# Autodesk Inventor assembly: FRC Fixed Field 2018_sldasm
(part 3 of 4)
- C:\Users\CAD\Documents\GitHub\FIRST-ROBOTICS-2018-5436-CAD\Field\FIRST Power Up Field CAD\Body_1193_sldprt.ipt
- C:\Users\CAD\Documents\GitHub\FIRST-ROBOTICS-2018-5436-CAD\Field\FIRST Power Up Field CAD\Body_1194_sldprt.ipt
- C:\Users\CAD\Documents\GitHub\FIRST-ROBOTICS-2018-5436-CAD\Field\FIRST Power Up Field CAD\Body_1195_sldprt.ipt
- C:\Users\CAD\Documents\GitHub\FIRST-ROBOTICS-2018-5436-CAD\Field\FIRST Power Up Field CAD\Body_1196_sldprt.ipt
- C:\Users\CAD\Documents\GitHub\FIRST-ROBOTICS-2018-5436-CAD\Field\FIRST Power Up Field CAD\Body_1197_sldprt.ipt
- C:\Users\CAD\Documents\GitHub\FIRST-ROBOTICS-2018-5436-CAD\Field\FIRST Power Up Field CAD\Body_1198_sldprt.ipt
- C:\Users\CAD\Documents\GitHub\FIRST-ROBOTICS-2018-5436-CAD\Field\FIRST Power Up Field CAD\Body_1199_sldprt.ipt
- C:\Users\CAD\Documents\GitHub\FIRST-ROBOTICS-2018-5436-CAD\Field\FIRST Power Up Field CAD\Body_1200_sldprt.ipt
- C:\Users\CAD\Documents\GitHub\FIRST-ROBOTICS-2018-5436-CAD\Field\FIRST Power Up Field CAD\Body_1201_sldprt.ipt
- C:\Users\CAD\Documents\GitHub\FIRST-ROBOTICS-2018-5436-CAD\Field\FIRST Power Up Field CAD\Body_1202_sldprt.ipt
- C:\Users\CAD\Documents\GitHub\FIRST-ROBOTICS-2018-5436-CAD\Field\FIRST Power Up Field CAD\Body_1203_sldprt.ipt
- C:\Users\CAD\Documents\GitHub\FIRST-ROBOTICS-2018-5436-CAD\Field\FIRST Power Up Field CAD\Body_1204_sldprt.ipt
- C:\Users\CAD\Documents\GitHub\FIRST-ROBOTICS-2018-5436-CAD\Field\FIRST Power Up Field CAD\Body_1205_sldprt.ipt
- C:\Users\CAD\Documents\GitHub\FIRST-ROBOTICS-2018-5436-CAD\Field\FIRST Power Up Field CAD\Body_1206_sldprt.ipt
- C:\Users\CAD\Documents\GitHub\FIRST-ROBOTICS-2018-5436-CAD\Field\FIRST Power Up Field CAD\Body_1207_sldprt.ipt
- C:\Users\CAD\Documents\GitHub\FIRST-ROBOTICS-2018-5436-CAD\Field\FIRST Power Up Field CAD\Body_1208_sldprt.ipt
- C:\Users\CAD\Documents\GitHub\FIRST-ROBOTICS-2018-5436-CAD\Field\FIRST Power Up Field CAD\Body_1209_sldprt.ipt
- C:\Users\CAD\Documents\GitHub\FIRST-ROBOTICS-2018-5436-CAD\Field\FIRST Power Up Field CAD\Body_1210_sldprt.ipt
- C:\Users\CAD\Documents\GitHub\FIRST-ROBOTICS-2018-5436-CAD\Field\FIRST Power Up Field CAD\Body_1211_sldprt.ipt
- C:\Users\CAD\Documents\GitHub\FIRST-ROBOTICS-2018-5436-CAD\Field\FIRST Power Up Field CAD\Body_1212_sldprt.ipt
- C:\Users\CAD\Documents\GitHub\FIRST-ROBOTICS-2018-5436-CAD\Field\FIRST Power Up Field CAD\Body_1213_sldprt.ipt
- C:\Users\CAD\Documents\GitHub\FIRST-ROBOTICS-2018-5436-CAD\Field\FIRST Power Up Field CAD\Body_1214_sldprt.ipt
- C:\Users\CAD\Documents\GitHub\FIRST-ROBOTICS-2018-5436-CAD\Field\FIRST Power Up Field CAD\Body_1215_sldprt.ipt
- C:\Users\CAD\Documents\GitHub\FIRST-ROBOTICS-2018-5436-CAD\Field\FIRST Power Up Field CAD\Body_1216_sldprt.ipt
- C:\Users\CAD\Documents\GitHub\FIRST-ROBOTICS-2018-5436-CAD\Field\FIRST Power Up Field CAD\Body_1217_sldprt.ipt
- C:\Users\CAD\Documents\GitHub\FIRST-ROBOTICS-2018-5436-CAD\Field\FIRST Power Up Field CAD\Body_1218_sldprt.ipt
- C:\Users\CAD\Documents\GitHub\FIRST-ROBOTICS-2018-5436-CAD\Field\FIRST Power Up Field CAD\Body_1219_sldprt.ipt
- C:\Users\CAD\Documents\GitHub\FIRST-ROBOTICS-2018-5436-CAD\Field\FIRST Power Up Field CAD\Body_1220_sldprt.ipt
- C:\Users\CAD\Documents\GitHub\FIRST-ROBOTICS-2018-5436-CAD\Field\FIRST Power Up Field CAD\Body_1221_sldprt.ipt
- C:\Users\CAD\Documents\GitHub\FIRST-ROBOTICS-2018-5436-CAD\Field\FIRST Power Up Field CAD\Body_1222_sldprt.ipt
- C:\Users\CAD\Documents\GitHub\FIRST-ROBOTICS-2018-5436-CAD\Field\FIRST Power Up Field CAD\Body_1223_sldprt.ipt
- C:\Users\CAD\Documents\GitHub\FIRST-ROBOTICS-2018-5436-CAD\Field\FIRST Power Up Field CAD\Body_1224_sldprt.ipt
- C:\Users\CAD\Documents\GitHub\FIRST-ROBOTICS-2018-5436-CAD\Field\FIRST Power Up Field CAD\Body_1225_sldprt.ipt
- C:\Users\CAD\Documents\GitHub\FIRST-ROBOTICS-2018-5436-CAD\Field\FIRST Power Up Field CAD\Body_1226_sldprt.ipt
- C:\Users\CAD\Documents\GitHub\FIRST-ROBOTICS-2018-5436-CAD\Field\FIRST Power Up Field CAD\Body_1227_sldprt.ipt
- C:\Users\CAD\Documents\GitHub\FIRST-ROBOTICS-2018-5436-CAD\Field\FIRST Power Up Field CAD\Body_1228_sldprt.ipt
- C:\Users\CAD\Documents\GitHub\FIRST-ROBOTICS-2018-5436-CAD\Field\FIRST Power Up Field CAD\Body_1229_sldprt.ipt
- C:\Users\CAD\Documents\GitHub\FIRST-ROBOTICS-2018-5436-CAD\Field\FIRST Power Up Field CAD\Body_1230_sldprt.ipt
- C:\Users\CAD\Documents\GitHub\FIRST-ROBOTICS-2018-5436-CAD\Field\FIRST Power Up Field CAD\Body_1231_sldprt.ipt
- C:\Users\CAD\Documents\GitHub\FIRST-ROBOTICS-2018-5436-CAD\Field\FIRST Power Up Field CAD\Body_1232_sldprt.ipt
- C:\Users\CAD\Documents\GitHub\FIRST-ROBOTICS-2018-5436-CAD\Field\FIRST Power Up Field CAD\Body_1233_sldprt.ipt
- C:\Users\CAD\Documents\GitHub\FIRST-ROBOTICS-2018-5436-CAD\Field\FIRST Power Up Field CAD\Body_1234_sldprt.ipt
- C:\Users\CAD\Documents\GitHub\FIRST-ROBOTICS-2018-5436-CAD\Field\FIRST Power Up Field CAD\Body_1235_sldprt.ipt
- C:\Users\CAD\Documents\GitHub\FIRST-ROBOTICS-2018-5436-CAD\Field\FIRST Power Up Field CAD\Body_1236_sldprt.ipt
- C:\Users\CAD\Documents\GitHub\FIRST-ROBOTICS-2018-5436-CAD\Field\FIRST Power Up Field CAD\Body_1237_sldprt.ipt
- C:\Users\CAD\Documents\GitHub\FIRST-ROBOTICS-2018-5436-CAD\Field\FIRST Power Up Field CAD\Body_1238_sldprt.ipt
- C:\Users\CAD\Documents\GitHub\FIRST-ROBOTICS-2018-5436-CAD\Field\FIRST Power Up Field CAD\Body_1239_sldprt.ipt
- C:\Users\CAD\Documents\GitHub\FIRST-ROBOTICS-2018-5436-CAD\Field\FIRST Power Up Field CAD\Body_1240_sldprt.ipt
- C:\Users\CAD\Documents\GitHub\FIRST-ROBOTICS-2018-5436-CAD\Field\FIRST Power Up Field CAD\Body_1241_sldprt.ipt
- C:\Users\CAD\Documents\GitHub\FIRST-ROBOTICS-2018-5436-CAD\Field\FIRST Power Up Field CAD\Body_1242_sldprt.ipt
- C:\Users\CAD\Documents\GitHub\FIRST-ROBOTICS-2018-5436-CAD\Field\FIRST Power Up Field CAD\Body_1243_sldprt.ipt
- C:\Users\CAD\Documents\GitHub\FIRST-ROBOTICS-2018-5436-CAD\Field\FIRST Power Up Field CAD\Body_1244_sldprt.ipt
- C:\Users\CAD\Documents\GitHub\FIRST-ROBOTICS-2018-5436-CAD\Field\FIRST Power Up Field CAD\Body_1245_sldprt.ipt
- C:\Users\CAD\Documents\GitHub\FIRST-ROBOTICS-2018-5436-CAD\Field\FIRST Power Up Field CAD\Body_1246_sldprt.ipt
- C:\Users\CAD\Documents\GitHub\FIRST-ROBOTICS-2018-5436-CAD\Field\FIRST Power Up Field CAD\Body_1247_sldprt.ipt
- C:\Users\CAD\Documents\GitHub\FIRST-ROBOTICS-2018-5436-CAD\Field\FIRST Power Up Field CAD\Body_1248_sldprt.ipt
- C:\Users\CAD\Documents\GitHub\FIRST-ROBOTICS-2018-5436-CAD\Field\FIRST Power Up Field CAD\Body_1249_sldprt.ipt
- C:\Users\CAD\Documents\GitHub\FIRST-ROBOTICS-2018-5436-CAD\Field\FIRST Power Up Field CAD\Body_1250_sldprt.ipt
- C:\Users\CAD\Documents\GitHub\FIRST-ROBOTICS-2018-5436-CAD\Field\FIRST Power Up Field CAD\Body_1251_sldprt.ipt
- C:\Users\CAD\Documents\GitHub\FIRST-ROBOTICS-2018-5436-CAD\Field\FIRST Power Up Field CAD\Body_1252_sldprt.ipt
- C:\Users\CAD\Documents\GitHub\FIRST-ROBOTICS-2018-5436-CAD\Field\FIRST Power Up Field CAD\Body_1253_sldprt.ipt
- C:\Users\CAD\Documents\GitHub\FIRST-ROBOTICS-2018-5436-CAD\Field\FIRST Power Up Field CAD\Body_1254_sldprt.ipt
- C:\Users\CAD\Documents\GitHub\FIRST-ROBOTICS-2018-5436-CAD\Field\FIRST Power Up Field CAD\Body_1255_sldprt.ipt
- C:\Users\CAD\Documents\GitHub\FIRST-ROBOTICS-2018-5436-CAD\Field\FIRST Power Up Field CAD\Body_1256_sldprt.ipt
- C:\Users\CAD\Documents\GitHub\FIRST-ROBOTICS-2018-5436-CAD\Field\FIRST Power Up Field CAD\Body_1257_sldprt.ipt
- C:\Users\CAD\Documents\GitHub\FIRST-ROBOTICS-2018-5436-CAD\Field\FIRST Power Up Field CAD\Body_1258_sldprt.ipt
- C:\Users\CAD\Documents\GitHub\FIRST-ROBOTICS-2018-5436-CAD\Field\FIRST Power Up Field CAD\Body_1259_sldprt.ipt
- C:\Users\CAD\Documents\GitHub\FIRST-ROBOTICS-2018-5436-CAD\Field\FIRST Power Up Field CAD\Body_1260_sldprt.ipt
- C:\Users\CAD\Documents\GitHub\FIRST-ROBOTICS-2018-5436-CAD\Field\FIRST Power Up Field CAD\Body_1261_sldprt.ipt
- C:\Users\CAD\Documents\GitHub\FIRST-ROBOTICS-2018-5436-CAD\Field\FIRST Power Up Field CAD\Body_1262_sldprt.ipt
- C:\Users\CAD\Documents\GitHub\FIRST-ROBOTICS-2018-5436-CAD\Field\FIRST Power Up Field CAD\Body_1263_sldprt.ipt
- C:\Users\CAD\Documents\GitHub\FIRST-ROBOTICS-2018-5436-CAD\Field\FIRST Power Up Field CAD\Body_1264_sldprt.ipt
- C:\Users\CAD\Documents\GitHub\FIRST-ROBOTICS-2018-5436-CAD\Field\FIRST Power Up Field CAD\Body_1265_sldprt.ipt
- C:\Users\CAD\Documents\GitHub\FIRST-ROBOTICS-2018-5436-CAD\Field\FIRST Power Up Field CAD\Body_1266_sldprt.ipt
- C:\Users\CAD\Documents\GitHub\FIRST-ROBOTICS-2018-5436-CAD\Field\FIRST Power Up Field CAD\Body_1267_sldprt.ipt
- C:\Users\CAD\Documents\GitHub\FIRST-ROBOTICS-2018-5436-CAD\Field\FIRST Power Up Field CAD\Body_1268_sldprt.ipt
- C:\Users\CAD\Documents\GitHub\FIRST-ROBOTICS-2018-5436-CAD\Field\FIRST Power Up Field CAD\Body_1269_sldprt.ipt
- C:\Users\CAD\Documents\GitHub\FIRST-ROBOTICS-2018-5436-CAD\Field\FIRST Power Up Field CAD\Body_1270_sldprt.ipt
- C:\Users\CAD\Documents\GitHub\FIRST-ROBOTICS-2018-5436-CAD\Field\FIRST Power Up Field CAD\Body_1271_sldprt.ipt
- C:\Users\CAD\Documents\GitHub\FIRST-ROBOTICS-2018-5436-CAD\Field\FIRST Power Up Field CAD\Body_1272_sldprt.ipt
- C:\Users\CAD\Documents\GitHub\FIRST-ROBOTICS-2018-5436-CAD\Field\FIRST Power Up Field CAD\Body_1273_sldprt.ipt
- C:\Users\CAD\Documents\GitHub\FIRST-ROBOTICS-2018-5436-CAD\Field\FIRST Power Up Field CAD\Body_1274_sldprt.ipt
- C:\Users\CAD\Documents\GitHub\FIRST-ROBOTICS-2018-5436-CAD\Field\FIRST Power Up Field CAD\Body_1275_sldprt.ipt
- C:\Users\CAD\Documents\GitHub\FIRST-ROBOTICS-2018-5436-CAD\Field\FIRST Power Up Field CAD\Body_1276_sldprt.ipt
- C:\Users\CAD\Documents\GitHub\FIRST-ROBOTICS-2018-5436-CAD\Field\FIRST Power Up Field CAD\Body_1277_sldprt.ipt
- C:\Users\CAD\Documents\GitHub\FIRST-ROBOTICS-2018-5436-CAD\Field\FIRST Power Up Field CAD\Body_1278_sldprt.ipt
- C:\Users\CAD\Documents\GitHub\FIRST-ROBOTICS-2018-5436-CAD\Field\FIRST Power Up Field CAD\Body_1279_sldprt.ipt
- C:\Users\CAD\Documents\GitHub\FIRST-ROBOTICS-2018-5436-CAD\Field\FIRST Power Up Field CAD\Body_1280_sldprt.ipt
- C:\Users\CAD\Documents\GitHub\FIRST-ROBOTICS-2018-5436-CAD\Field\FIRST Power Up Field CAD\Body_1281_sldprt.ipt
- C:\Users\CAD\Documents\GitHub\FIRST-ROBOTICS-2018-5436-CAD\Field\FIRST Power Up Field CAD\Body_1282_sldprt.ipt
- C:\Users\CAD\Documents\GitHub\FIRST-ROBOTICS-2018-5436-CAD\Field\FIRST Power Up Field CAD\Body_1283_sldprt.ipt
- C:\Users\CAD\Documents\GitHub\FIRST-ROBOTICS-2018-5436-CAD\Field\FIRST Power Up Field CAD\Body_1284_sldprt.ipt
- C:\Users\CAD\Documents\GitHub\FIRST-ROBOTICS-2018-5436-CAD\Field\FIRST Power Up Field CAD\Body_1285_sldprt.ipt
- C:\Users\CAD\Documents\GitHub\FIRST-ROBOTICS-2018-5436-CAD\Field\FIRST Power Up Field CAD\Body_1286_sldprt.ipt
- C:\Users\CAD\Documents\GitHub\FIRST-ROBOTICS-2018-5436-CAD\Field\FIRST Power Up Field CAD\Body_1287_sldprt.ipt
- C:\Users\CAD\Documents\GitHub\FIRST-ROBOTICS-2018-5436-CAD\Field\FIRST Power Up Field CAD\Body_1288_sldprt.ipt
- C:\Users\CAD\Documents\GitHub\FIRST-ROBOTICS-2018-5436-CAD\Field\FIRST Power Up Field CAD\Body_1289_sldprt.ipt
- C:\Users\CAD\Documents\GitHub\FIRST-ROBOTICS-2018-5436-CAD\Field\FIRST Power Up Field CAD\Body_1290_sldprt.ipt
- C:\Users\CAD\Documents\GitHub\FIRST-ROBOTICS-2018-5436-CAD\Field\FIRST Power Up Field CAD\Body_1291_sldprt.ipt
- C:\Users\CAD\Documents\GitHub\FIRST-ROBOTICS-2018-5436-CAD\Field\FIRST Power Up Field CAD\Body_1292_sldprt.ipt
- C:\Users\CAD\Documents\GitHub\FIRST-ROBOTICS-2018-5436-CAD\Field\FIRST Power Up Field CAD\Body_1293_sldprt.ipt
- C:\Users\CAD\Documents\GitHub\FIRST-ROBOTICS-2018-5436-CAD\Field\FIRST Power Up Field CAD\Body_1294_sldprt.ipt
- C:\Users\CAD\Documents\GitHub\FIRST-ROBOTICS-2018-5436-CAD\Field\FIRST Power Up Field CAD\Body_1295_sldprt.ipt
- C:\Users\CAD\Documents\GitHub\FIRST-ROBOTICS-2018-5436-CAD\Field\FIRST Power Up Field CAD\Body_1296_sldprt.ipt
- C:\Users\CAD\Documents\GitHub\FIRST-ROBOTICS-2018-5436-CAD\Field\FIRST Power Up Field CAD\Body_1297_sldprt.ipt
- C:\Users\CAD\Documents\GitHub\FIRST-ROBOTICS-2018-5436-CAD\Field\FIRST Power Up Field CAD\Body_1298_sldprt.ipt
- C:\Users\CAD\Documents\GitHub\FIRST-ROBOTICS-2018-5436-CAD\Field\FIRST Power Up Field CAD\Body_1299_sldprt.ipt
- C:\Users\CAD\Documents\GitHub\FIRST-ROBOTICS-2018-5436-CAD\Field\FIRST Power Up Field CAD\Body_1300_sldprt.ipt
- C:\Users\CAD\Documents\GitHub\FIRST-ROBOTICS-2018-5436-CAD\Field\FIRST Power Up Field CAD\Body_1301_sldprt.ipt
- C:\Users\CAD\Documents\GitHub\FIRST-ROBOTICS-2018-5436-CAD\Field\FIRST Power Up Field CAD\Body_1302_sldprt.ipt
- C:\Users\CAD\Documents\GitHub\FIRST-ROBOTICS-2018-5436-CAD\Field\FIRST Power Up Field CAD\Body_1303_sldprt.ipt
- C:\Users\CAD\Documents\GitHub\FIRST-ROBOTICS-2018-5436-CAD\Field\FIRST Power Up Field CAD\Body_1304_sldprt.ipt
- C:\Users\CAD\Documents\GitHub\FIRST-ROBOTICS-2018-5436-CAD\Field\FIRST Power Up Field CAD\Body_1305_sldprt.ipt
- C:\Users\CAD\Documents\GitHub\FIRST-ROBOTICS-2018-5436-CAD\Field\FIRST Power Up Field CAD\Body_1306_sldprt.ipt
- C:\Users\CAD\Documents\GitHub\FIRST-ROBOTICS-2018-5436-CAD\Field\FIRST Power Up Field CAD\Body_1307_sldprt.ipt
- C:\Users\CAD\Documents\GitHub\FIRST-ROBOTICS-2018-5436-CAD\Field\FIRST Power Up Field CAD\Body_1308_sldprt.ipt
- C:\Users\CAD\Documents\GitHub\FIRST-ROBOTICS-2018-5436-CAD\Field\FIRST Power Up Field CAD\Body_1309_sldprt.ipt
- C:\Users\CAD\Documents\GitHub\FIRST-ROBOTICS-2018-5436-CAD\Field\FIRST Power Up Field CAD\Body_1310_sldprt.ipt
- C:\Users\CAD\Documents\GitHub\FIRST-ROBOTICS-2018-5436-CAD\Field\FIRST Power Up Field CAD\Body_1311_sldprt.ipt
- C:\Users\CAD\Documents\GitHub\FIRST-ROBOTICS-2018-5436-CAD\Field\FIRST Power Up Field CAD\Body_1312_sldprt.ipt
- C:\Users\CAD\Documents\GitHub\FIRST-ROBOTICS-2018-5436-CAD\Field\FIRST Power Up Field CAD\Body_1313_sldprt.ipt
- C:\Users\CAD\Documents\GitHub\FIRST-ROBOTICS-2018-5436-CAD\Field\FIRST Power Up Field CAD\Body_1314_sldprt.ipt
- C:\Users\CAD\Documents\GitHub\FIRST-ROBOTICS-2018-5436-CAD\Field\FIRST Power Up Field CAD\Body_1315_sldprt.ipt
- C:\Users\CAD\Documents\GitHub\FIRST-ROBOTICS-2018-5436-CAD\Field\FIRST Power Up Field CAD\Body_1316_sldprt.ipt
- C:\Users\CAD\Documents\GitHub\FIRST-ROBOTICS-2018-5436-CAD\Field\FIRST Power Up Field CAD\Body_1317_sldprt.ipt
- C:\Users\CAD\Documents\GitHub\FIRST-ROBOTICS-2018-5436-CAD\Field\FIRST Power Up Field CAD\Body_1318_sldprt.ipt
- C:\Users\CAD\Documents\GitHub\FIRST-ROBOTICS-2018-5436-CAD\Field\FIRST Power Up Field CAD\Body_1319_sldprt.ipt
- C:\Users\CAD\Documents\GitHub\FIRST-ROBOTICS-2018-5436-CAD\Field\FIRST Power Up Field CAD\Body_1320_sldprt.ipt
- C:\Users\CAD\Documents\GitHub\FIRST-ROBOTICS-2018-5436-CAD\Field\FIRST Power Up Field CAD\Body_1321_sldprt.ipt
- C:\Users\CAD\Documents\GitHub\FIRST-ROBOTICS-2018-5436-CAD\Field\FIRST Power Up Field CAD\Body_1322_sldprt.ipt
- C:\Users\CAD\Documents\GitHub\FIRST-ROBOTICS-2018-5436-CAD\Field\FIRST Power Up Field CAD\Body_1323_sldprt.ipt
- C:\Users\CAD\Documents\GitHub\FIRST-ROBOTICS-2018-5436-CAD\Field\FIRST Power Up Field CAD\Body_1324_sldprt.ipt
- C:\Users\CAD\Documents\GitHub\FIRST-ROBOTICS-2018-5436-CAD\Field\FIRST Power Up Field CAD\Body_1325_sldprt.ipt
- C:\Users\CAD\Documents\GitHub\FIRST-ROBOTICS-2018-5436-CAD\Field\FIRST Power Up Field CAD\Body_1326_sldprt.ipt
- C:\Users\CAD\Documents\GitHub\FIRST-ROBOTICS-2018-5436-CAD\Field\FIRST Power Up Field CAD\Body_1327_sldprt.ipt
- C:\Users\CAD\Documents\GitHub\FIRST-ROBOTICS-2018-5436-CAD\Field\FIRST Power Up Field CAD\Body_1328_sldprt.ipt
- C:\Users\CAD\Documents\GitHub\FIRST-ROBOTICS-2018-5436-CAD\Field\FIRST Power Up Field CAD\Body_1329_sldprt.ipt
- C:\Users\CAD\Documents\GitHub\FIRST-ROBOTICS-2018-5436-CAD\Field\FIRST Power Up Field CAD\Body_1330_sldprt.ipt
- C:\Users\CAD\Documents\GitHub\FIRST-ROBOTICS-2018-5436-CAD\Field\FIRST Power Up Field CAD\Body_1331_sldprt.ipt
- C:\Users\CAD\Documents\GitHub\FIRST-ROBOTICS-2018-5436-CAD\Field\FIRST Power Up Field CAD\Body_1332_sldprt.ipt
- C:\Users\CAD\Documents\GitHub\FIRST-ROBOTICS-2018-5436-CAD\Field\FIRST Power Up Field CAD\Body_1333_sldprt.ipt
- C:\Users\CAD\Documents\GitHub\FIRST-ROBOTICS-2018-5436-CAD\Field\FIRST Power Up Field CAD\Body_1334_sldprt.ipt
- C:\Users\CAD\Documents\GitHub\FIRST-ROBOTICS-2018-5436-CAD\Field\FIRST Power Up Field CAD\Body_1335_sldprt.ipt
- C:\Users\CAD\Documents\GitHub\FIRST-ROBOTICS-2018-5436-CAD\Field\FIRST Power Up Field CAD\Body_1336_sldprt.ipt
- C:\Users\CAD\Documents\GitHub\FIRST-ROBOTICS-2018-5436-CAD\Field\FIRST Power Up Field CAD\Body_1337_sldprt.ipt
- C:\Users\CAD\Documents\GitHub\FIRST-ROBOTICS-2018-5436-CAD\Field\FIRST Power Up Field CAD\Body_1338_sldprt.ipt
- C:\Users\CAD\Documents\GitHub\FIRST-ROBOTICS-2018-5436-CAD\Field\FIRST Power Up Field CAD\Body_1339_sldprt.ipt
- C:\Users\CAD\Documents\GitHub\FIRST-ROBOTICS-2018-5436-CAD\Field\FIRST Power Up Field CAD\Body_1340_sldprt.ipt
- C:\Users\CAD\Documents\GitHub\FIRST-ROBOTICS-2018-5436-CAD\Field\FIRST Power Up Field CAD\Body_1341_sldprt.ipt
- C:\Users\CAD\Documents\GitHub\FIRST-ROBOTICS-2018-5436-CAD\Field\FIRST Power Up Field CAD\Body_1342_sldprt.ipt
- C:\Users\CAD\Documents\GitHub\FIRST-ROBOTICS-2018-5436-CAD\Field\FIRST Power Up Field CAD\Body_1343_sldprt.ipt
- C:\Users\CAD\Documents\GitHub\FIRST-ROBOTICS-2018-5436-CAD\Field\FIRST Power Up Field CAD\Body_1344_sldprt.ipt
- C:\Users\CAD\Documents\GitHub\FIRST-ROBOTICS-2018-5436-CAD\Field\FIRST Power Up Field CAD\Body_1345_sldprt.ipt
- C:\Users\CAD\Documents\GitHub\FIRST-ROBOTICS-2018-5436-CAD\Field\FIRST Power Up Field CAD\Body_1346_sldprt.ipt
- C:\Users\CAD\Documents\GitHub\FIRST-ROBOTICS-2018-5436-CAD\Field\FIRST Power Up Field CAD\Body_1347_sldprt.ipt
- C:\Users\CAD\Documents\GitHub\FIRST-ROBOTICS-2018-5436-CAD\Field\FIRST Power Up Field CAD\Body_1348_sldprt.ipt
- C:\Users\CAD\Documents\GitHub\FIRST-ROBOTICS-2018-5436-CAD\Field\FIRST Power Up Field CAD\Body_1349_sldprt.ipt
- C:\Users\CAD\Documents\GitHub\FIRST-ROBOTICS-2018-5436-CAD\Field\FIRST Power Up Field CAD\Body_1350_sldprt.ipt
- C:\Users\CAD\Documents\GitHub\FIRST-ROBOTICS-2018-5436-CAD\Field\FIRST Power Up Field CAD\Body_1351_sldprt.ipt
- C:\Users\CAD\Documents\GitHub\FIRST-ROBOTICS-2018-5436-CAD\Field\FIRST Power Up Field CAD\Body_1352_sldprt.ipt
- C:\Users\CAD\Documents\GitHub\FIRST-ROBOTICS-2018-5436-CAD\Field\FIRST Power Up Field CAD\Body_1353_sldprt.ipt
- C:\Users\CAD\Documents\GitHub\FIRST-ROBOTICS-2018-5436-CAD\Field\FIRST Power Up Field CAD\Body_1354_sldprt.ipt
- C:\Users\CAD\Documents\GitHub\FIRST-ROBOTICS-2018-5436-CAD\Field\FIRST Power Up Field CAD\Body_1355_sldprt.ipt
- C:\Users\CAD\Documents\GitHub\FIRST-ROBOTICS-2018-5436-CAD\Field\FIRST Power Up Field CAD\Body_1356_sldprt.ipt
- C:\Users\CAD\Documents\GitHub\FIRST-ROBOTICS-2018-5436-CAD\Field\FIRST Power Up Field CAD\Body_1357_sldprt.ipt
- C:\Users\CAD\Documents\GitHub\FIRST-ROBOTICS-2018-5436-CAD\Field\FIRST Power Up Field CAD\Body_1358_sldprt.ipt
- C:\Users\CAD\Documents\GitHub\FIRST-ROBOTICS-2018-5436-CAD\Field\FIRST Power Up Field CAD\Body_1359_sldprt.ipt
- C:\Users\CAD\Documents\GitHub\FIRST-ROBOTICS-2018-5436-CAD\Field\FIRST Power Up Field CAD\Body_1360_sldprt.ipt
- C:\Users\CAD\Documents\GitHub\FIRST-ROBOTICS-2018-5436-CAD\Field\FIRST Power Up Field CAD\Body_1361_sldprt.ipt
- C:\Users\CAD\Documents\GitHub\FIRST-ROBOTICS-2018-5436-CAD\Field\FIRST Power Up Field CAD\Body_1362_sldprt.ipt
- C:\Users\CAD\Documents\GitHub\FIRST-ROBOTICS-2018-5436-CAD\Field\FIRST Power Up Field CAD\Body_1363_sldprt.ipt
- C:\Users\CAD\Documents\GitHub\FIRST-ROBOTICS-2018-5436-CAD\Field\FIRST Power Up Field CAD\Body_1364_sldprt.ipt
- C:\Users\CAD\Documents\GitHub\FIRST-ROBOTICS-2018-5436-CAD\Field\FIRST Power Up Field CAD\Body_1365_sldprt.ipt
- C:\Users\CAD\Documents\GitHub\FIRST-ROBOTICS-2018-5436-CAD\Field\FIRST Power Up Field CAD\Body_1366_sldprt.ipt
- C:\Users\CAD\Documents\GitHub\FIRST-ROBOTICS-2018-5436-CAD\Field\FIRST Power Up Field CAD\Body_1367_sldprt.ipt
- C:\Users\CAD\Documents\GitHub\FIRST-ROBOTICS-2018-5436-CAD\Field\FIRST Power Up Field CAD\Body_1368_sldprt.ipt
- C:\Users\CAD\Documents\GitHub\FIRST-ROBOTICS-2018-5436-CAD\Field\FIRST Power Up Field CAD\Body_1369_sldprt.ipt
- C:\Users\CAD\Documents\GitHub\FIRST-ROBOTICS-2018-5436-CAD\Field\FIRST Power Up Field CAD\Body_1370_sldprt.ipt
- C:\Users\CAD\Documents\GitHub\FIRST-ROBOTICS-2018-5436-CAD\Field\FIRST Power Up Field CAD\Body_1371_sldprt.ipt
- C:\Users\CAD\Documents\GitHub\FIRST-ROBOTICS-2018-5436-CAD\Field\FIRST Power Up Field CAD\Body_1372_sldprt.ipt
- C:\Users\CAD\Documents\GitHub\FIRST-ROBOTICS-2018-5436-CAD\Field\FIRST Power Up Field CAD\Body_1373_sldprt.ipt
- C:\Users\CAD\Documents\GitHub\FIRST-ROBOTICS-2018-5436-CAD\Field\FIRST Power Up Field CAD\Body_1374_sldprt.ipt
- C:\Users\CAD\Documents\GitHub\FIRST-ROBOTICS-2018-5436-CAD\Field\FIRST Power Up Field CAD\Body_1375_sldprt.ipt
- C:\Users\CAD\Documents\GitHub\FIRST-ROBOTICS-2018-5436-CAD\Field\FIRST Power Up Field CAD\Body_1376_sldprt.ipt
- C:\Users\CAD\Documents\GitHub\FIRST-ROBOTICS-2018-5436-CAD\Field\FIRST Power Up Field CAD\Body_1377_sldprt.ipt
- C:\Users\CAD\Documents\GitHub\FIRST-ROBOTICS-2018-5436-CAD\Field\FIRST Power Up Field CAD\Body_1378_sldprt.ipt
- C:\Users\CAD\Documents\GitHub\FIRST-ROBOTICS-2018-5436-CAD\Field\FIRST Power Up Field CAD\Body_1379_sldprt.ipt
- C:\Users\CAD\Documents\GitHub\FIRST-ROBOTICS-2018-5436-CAD\Field\FIRST Power Up Field CAD\Body_1380_sldprt.ipt
- C:\Users\CAD\Documents\GitHub\FIRST-ROBOTICS-2018-5436-CAD\Field\FIRST Power Up Field CAD\Body_1381_sldprt.ipt
- C:\Users\CAD\Documents\GitHub\FIRST-ROBOTICS-2018-5436-CAD\Field\FIRST Power Up Field CAD\Body_1382_sldprt.ipt
- C:\Users\CAD\Documents\GitHub\FIRST-ROBOTICS-2018-5436-CAD\Field\FIRST Power Up Field CAD\Body_1383_sldprt.ipt
- C:\Users\CAD\Documents\GitHub\FIRST-ROBOTICS-2018-5436-CAD\Field\FIRST Power Up Field CAD\Body_1384_sldprt.ipt
- C:\Users\CAD\Documents\GitHub\FIRST-ROBOTICS-2018-5436-CAD\Field\FIRST Power Up Field CAD\Body_1385_sldprt.ipt
- C:\Users\CAD\Documents\GitHub\FIRST-ROBOTICS-2018-5436-CAD\Field\FIRST Power Up Field CAD\Body_1386_sldprt.ipt
- C:\Users\CAD\Documents\GitHub\FIRST-ROBOTICS-2018-5436-CAD\Field\FIRST Power Up Field CAD\Body_1387_sldprt.ipt
- C:\Users\CAD\Documents\GitHub\FIRST-ROBOTICS-2018-5436-CAD\Field\FIRST Power Up Field CAD\Body_1388_sldprt.ipt
- C:\Users\CAD\Documents\GitHub\FIRST-ROBOTICS-2018-5436-CAD\Field\FIRST Power Up Field CAD\Body_1389_sldprt.ipt
- C:\Users\CAD\Documents\GitHub\FIRST-ROBOTICS-2018-5436-CAD\Field\FIRST Power Up Field CAD\Body_1390_sldprt.ipt
- C:\Users\CAD\Documents\GitHub\FIRST-ROBOTICS-2018-5436-CAD\Field\FIRST Power Up Field CAD\Body_1391_sldprt.ipt
- C:\Users\CAD\Documents\GitHub\FIRST-ROBOTICS-2018-5436-CAD\Field\FIRST Power Up Field CAD\Body_1392_sldprt.ipt
- C:\Users\CAD\Documents\GitHub\FIRST-ROBOTICS-2018-5436-CAD\Field\FIRST Power Up Field CAD\Body_1393_sldprt.ipt
- C:\Users\CAD\Documents\GitHub\FIRST-ROBOTICS-2018-5436-CAD\Field\FIRST Power Up Field CAD\Body_1394_sldprt.ipt
- C:\Users\CAD\Documents\GitHub\FIRST-ROBOTICS-2018-5436-CAD\Field\FIRST Power Up Field CAD\Body_1395_sldprt.ipt
- C:\Users\CAD\Documents\GitHub\FIRST-ROBOTICS-2018-5436-CAD\Field\FIRST Power Up Field CAD\Body_1396_sldprt.ipt
- C:\Users\CAD\Documents\GitHub\FIRST-ROBOTICS-2018-5436-CAD\Field\FIRST Power Up Field CAD\Body_1397_sldprt.ipt
- C:\Users\CAD\Documents\GitHub\FIRST-ROBOTICS-2018-5436-CAD\Field\FIRST Power Up Field CAD\Body_1398_sldprt.ipt
- C:\Users\CAD\Documents\GitHub\FIRST-ROBOTICS-2018-5436-CAD\Field\FIRST Power Up Field CAD\Body_1399_sldprt.ipt
- C:\Users\CAD\Documents\GitHub\FIRST-ROBOTICS-2018-5436-CAD\Field\FIRST Power Up Field CAD\Body_1400_sldprt.ipt
- C:\Users\CAD\Documents\GitHub\FIRST-ROBOTICS-2018-5436-CAD\Field\FIRST Power Up Field CAD\Body_1401_sldprt.ipt
- C:\Users\CAD\Documents\GitHub\FIRST-ROBOTICS-2018-5436-CAD\Field\FIRST Power Up Field CAD\Body_1402_sldprt.ipt
- C:\Users\CAD\Documents\GitHub\FIRST-ROBOTICS-2018-5436-CAD\Field\FIRST Power Up Field CAD\Body_1403_sldprt.ipt
- C:\Users\CAD\Documents\GitHub\FIRST-ROBOTICS-2018-5436-CAD\Field\FIRST Power Up Field CAD\Body_1404_sldprt.ipt
- C:\Users\CAD\Documents\GitHub\FIRST-ROBOTICS-2018-5436-CAD\Field\FIRST Power Up Field CAD\Body_1405_sldprt.ipt
- C:\Users\CAD\Documents\GitHub\FIRST-ROBOTICS-2018-5436-CAD\Field\FIRST Power Up Field CAD\Body_1406_sldprt.ipt
- C:\Users\CAD\Documents\GitHub\FIRST-ROBOTICS-2018-5436-CAD\Field\FIRST Power Up Field CAD\Body_1407_sldprt.ipt
- C:\Users\CAD\Documents\GitHub\FIRST-ROBOTICS-2018-5436-CAD\Field\FIRST Power Up Field CAD\Body_1408_sldprt.ipt
- C:\Users\CAD\Documents\GitHub\FIRST-ROBOTICS-2018-5436-CAD\Field\FIRST Power Up Field CAD\Body_1409_sldprt.ipt
- C:\Users\CAD\Documents\GitHub\FIRST-ROBOTICS-2018-5436-CAD\Field\FIRST Power Up Field CAD\Body_1410_sldprt.ipt
- C:\Users\CAD\Documents\GitHub\FIRST-ROBOTICS-2018-5436-CAD\Field\FIRST Power Up Field CAD\Body_1411_sldprt.ipt
- C:\Users\CAD\Documents\GitHub\FIRST-ROBOTICS-2018-5436-CAD\Field\FIRST Power Up Field CAD\Body_1412_sldprt.ipt
- C:\Users\CAD\Documents\GitHub\FIRST-ROBOTICS-2018-5436-CAD\Field\FIRST Power Up Field CAD\Body_1413_sldprt.ipt
- C:\Users\CAD\Documents\GitHub\FIRST-ROBOTICS-2018-5436-CAD\Field\FIRST Power Up Field CAD\Body_1414_sldprt.ipt
- C:\Users\CAD\Documents\GitHub\FIRST-ROBOTICS-2018-5436-CAD\Field\FIRST Power Up Field CAD\Body_1415_sldprt.ipt
- C:\Users\CAD\Documents\GitHub\FIRST-ROBOTICS-2018-5436-CAD\Field\FIRST Power Up Field CAD\Body_1416_sldprt.ipt
- C:\Users\CAD\Documents\GitHub\FIRST-ROBOTICS-2018-5436-CAD\Field\FIRST Power Up Field CAD\Body_1417_sldprt.ipt
- C:\Users\CAD\Documents\GitHub\FIRST-ROBOTICS-2018-5436-CAD\Field\FIRST Power Up Field CAD\Body_1418_sldprt.ipt
- C:\Users\CAD\Documents\GitHub\FIRST-ROBOTICS-2018-5436-CAD\Field\FIRST Power Up Field CAD\Body_1419_sldprt.ipt
- C:\Users\CAD\Documents\GitHub\FIRST-ROBOTICS-2018-5436-CAD\Field\FIRST Power Up Field CAD\Body_1420_sldprt.ipt
- C:\Users\CAD\Documents\GitHub\FIRST-ROBOTICS-2018-5436-CAD\Field\FIRST Power Up Field CAD\Body_1421_sldprt.ipt
- C:\Users\CAD\Documents\GitHub\FIRST-ROBOTICS-2018-5436-CAD\Field\FIRST Power Up Field CAD\Body_1422_sldprt.ipt
- C:\Users\CAD\Documents\GitHub\FIRST-ROBOTICS-2018-5436-CAD\Field\FIRST Power Up Field CAD\Body_1423_sldprt.ipt
- C:\Users\CAD\Documents\GitHub\FIRST-ROBOTICS-2018-5436-CAD\Field\FIRST Power Up Field CAD\Body_1424_sldprt.ipt
- C:\Users\CAD\Documents\GitHub\FIRST-ROBOTICS-2018-5436-CAD\Field\FIRST Power Up Field CAD\Body_1425_sldprt.ipt
- C:\Users\CAD\Documents\GitHub\FIRST-ROBOTICS-2018-5436-CAD\Field\FIRST Power Up Field CAD\Body_1426_sldprt.ipt
- C:\Users\CAD\Documents\GitHub\FIRST-ROBOTICS-2018-5436-CAD\Field\FIRST Power Up Field CAD\Body_1427_sldprt.ipt
- C:\Users\CAD\Documents\GitHub\FIRST-ROBOTICS-2018-5436-CAD\Field\FIRST Power Up Field CAD\Body_1428_sldprt.ipt
- C:\Users\CAD\Documents\GitHub\FIRST-ROBOTICS-2018-5436-CAD\Field\FIRST Power Up Field CAD\Body_1429_sldprt.ipt
- C:\Users\CAD\Documents\GitHub\FIRST-ROBOTICS-2018-5436-CAD\Field\FIRST Power Up Field CAD\Body_1430_sldprt.ipt
- C:\Users\CAD\Documents\GitHub\FIRST-ROBOTICS-2018-5436-CAD\Field\FIRST Power Up Field CAD\Body_1431_sldprt.ipt
- C:\Users\CAD\Documents\GitHub\FIRST-ROBOTICS-2018-5436-CAD\Field\FIRST Power Up Field CAD\Body_1432_sldprt.ipt
- C:\Users\CAD\Documents\GitHub\FIRST-ROBOTICS-2018-5436-CAD\Field\FIRST Power Up Field CAD\Body_1433_sldprt.ipt
- C:\Users\CAD\Documents\GitHub\FIRST-ROBOTICS-2018-5436-CAD\Field\FIRST Power Up Field CAD\Body_1434_sldprt.ipt
- C:\Users\CAD\Documents\GitHub\FIRST-ROBOTICS-2018-5436-CAD\Field\FIRST Power Up Field CAD\Body_1435_sldprt.ipt
- C:\Users\CAD\Documents\GitHub\FIRST-ROBOTICS-2018-5436-CAD\Field\FIRST Power Up Field CAD\Body_1436_sldprt.ipt
- C:\Users\CAD\Documents\GitHub\FIRST-ROBOTICS-2018-5436-CAD\Field\FIRST Power Up Field CAD\Body_1437_sldprt.ipt
- C:\Users\CAD\Documents\GitHub\FIRST-ROBOTICS-2018-5436-CAD\Field\FIRST Power Up Field CAD\Body_1438_sldprt.ipt
- C:\Users\CAD\Documents\GitHub\FIRST-ROBOTICS-2018-5436-CAD\Field\FIRST Power Up Field CAD\Body_1439_sldprt.ipt
- C:\Users\CAD\Documents\GitHub\FIRST-ROBOTICS-2018-5436-CAD\Field\FIRST Power Up Field CAD\Body_1440_sldprt.ipt
- C:\Users\CAD\Documents\GitHub\FIRST-ROBOTICS-2018-5436-CAD\Field\FIRST Power Up Field CAD\Body_1441_sldprt.ipt
- C:\Users\CAD\Documents\GitHub\FIRST-ROBOTICS-2018-5436-CAD\Field\FIRST Power Up Field CAD\Body_1442_sldprt.ipt
- C:\Users\CAD\Documents\GitHub\FIRST-ROBOTICS-2018-5436-CAD\Field\FIRST Power Up Field CAD\Body_1443_sldprt.ipt
- C:\Users\CAD\Documents\GitHub\FIRST-ROBOTICS-2018-5436-CAD\Field\FIRST Power Up Field CAD\Body_1444_sldprt.ipt
- C:\Users\CAD\Documents\GitHub\FIRST-ROBOTICS-2018-5436-CAD\Field\FIRST Power Up Field CAD\Body_1445_sldprt.ipt
- C:\Users\CAD\Documents\GitHub\FIRST-ROBOTICS-2018-5436-CAD\Field\FIRST Power Up Field CAD\Body_1446_sldprt.ipt
- C:\Users\CAD\Documents\GitHub\FIRST-ROBOTICS-2018-5436-CAD\Field\FIRST Power Up Field CAD\Body_1447_sldprt.ipt
- C:\Users\CAD\Documents\GitHub\FIRST-ROBOTICS-2018-5436-CAD\Field\FIRST Power Up Field CAD\Body_1448_sldprt.ipt
- C:\Users\CAD\Documents\GitHub\FIRST-ROBOTICS-2018-5436-CAD\Field\FIRST Power Up Field CAD\Body_1449_sldprt.ipt
- C:\Users\CAD\Documents\GitHub\FIRST-ROBOTICS-2018-5436-CAD\Field\FIRST Power Up Field CAD\Body_1450_sldprt.ipt
- C:\Users\CAD\Documents\GitHub\FIRST-ROBOTICS-2018-5436-CAD\Field\FIRST Power Up Field CAD\Body_1451_sldprt.ipt
- C:\Users\CAD\Documents\GitHub\FIRST-ROBOTICS-2018-5436-CAD\Field\FIRST Power Up Field CAD\Body_1452_sldprt.ipt
- C:\Users\CAD\Documents\GitHub\FIRST-ROBOTICS-2018-5436-CAD\Field\FIRST Power Up Field CAD\Body_1453_sldprt.ipt
- C:\Users\CAD\Documents\GitHub\FIRST-ROBOTICS-2018-5436-CAD\Field\FIRST Power Up Field CAD\Body_1454_sldprt.ipt
- C:\Users\CAD\Documents\GitHub\FIRST-ROBOTICS-2018-5436-CAD\Field\FIRST Power Up Field CAD\Body_1455_sldprt.ipt
- C:\Users\CAD\Documents\GitHub\FIRST-ROBOTICS-2018-5436-CAD\Field\FIRST Power Up Field CAD\Body_1456_sldprt.ipt
- C:\Users\CAD\Documents\GitHub\FIRST-ROBOTICS-2018-5436-CAD\Field\FIRST Power Up Field CAD\Body_1457_sldprt.ipt
- C:\Users\CAD\Documents\GitHub\FIRST-ROBOTICS-2018-5436-CAD\Field\FIRST Power Up Field CAD\Body_1458_sldprt.ipt
- C:\Users\CAD\Documents\GitHub\FIRST-ROBOTICS-2018-5436-CAD\Field\FIRST Power Up Field CAD\Body_1459_sldprt.ipt
- C:\Users\CAD\Documents\GitHub\FIRST-ROBOTICS-2018-5436-CAD\Field\FIRST Power Up Field CAD\Body_1460_sldprt.ipt
- C:\Users\CAD\Documents\GitHub\FIRST-ROBOTICS-2018-5436-CAD\Field\FIRST Power Up Field CAD\Body_1461_sldprt.ipt
- C:\Users\CAD\Documents\GitHub\FIRST-ROBOTICS-2018-5436-CAD\Field\FIRST Power Up Field CAD\Body_1462_sldprt.ipt
- C:\Users\CAD\Documents\GitHub\FIRST-ROBOTICS-2018-5436-CAD\Field\FIRST Power Up Field CAD\Body_1463_sldprt.ipt
- C:\Users\CAD\Documents\GitHub\FIRST-ROBOTICS-2018-5436-CAD\Field\FIRST Power Up Field CAD\Body_1464_sldprt.ipt
- C:\Users\CAD\Documents\GitHub\FIRST-ROBOTICS-2018-5436-CAD\Field\FIRST Power Up Field CAD\Body_1465_sldprt.ipt
- C:\Users\CAD\Documents\GitHub\FIRST-ROBOTICS-2018-5436-CAD\Field\FIRST Power Up Field CAD\Body_1466_sldprt.ipt
## Components (942 placed, 942 different names)
1. Body_525_sldprt_1001
2. Body_526_sldprt_1002
3. Body_527_sldprt_1003
4. Body_528_sldprt_1004
5. Body_529_sldprt_1005
6. Body_530_sldprt_1006
7. Body_531_sldprt_1007
8. Body_532_sldprt_1008
9. Body_533_sldprt_1009
10. Body_534_sldprt_1010
11. Body_535_sldprt_1011
12. Body_536_sldprt_1012
13. Body_537_sldprt_1013
14. Body_538_sldprt_1014
15. Body_539_sldprt_1015
16. Body_540_sldprt_1016
17. Body_541_sldprt_1017
18. Body_542_sldprt_1018
19. Body_543_sldprt_1019
20. Body_544_sldprt_1020
21. Body_545_sldprt_1021
22. Body_546_sldprt_1022
23. Body_547_sldprt_1023
24. Body_548_sldprt_1024
25. Body_549_sldprt_1025
26. Body_550_sldprt_1026
27. Body_551_sldprt_1027
28. Body_552_sldprt_1028
29. Body_553_sldprt_1029
30. Body_554_sldprt_1030
31. Body_555_sldprt_1031
32. Body_556_sldprt_1032
33. Body_557_sldprt_1033
34. Body_558_sldprt_1034
35. Body_559_sldprt_1035
36. Body_560_sldprt_1036
37. Body_561_sldprt_1037
38. Body_562_sldprt_1038
39. Body_563_sldprt_1039
40. Body_564_sldprt_1040
41. Body_565_sldprt_1041
42. Body_566_sldprt_1042
43. Body_567_sldprt_1043
44. Body_568_sldprt_1044
45. Body_569_sldprt_1045
46. Body_570_sldprt_1046
47. Body_571_sldprt_1047
48. Body_572_sldprt_1048
49. Body_573_sldprt_1049
50. Body_574_sldprt_1050
51. Body_575_sldprt_1051
52. Body_576_sldprt_1052
53. Body_577_sldprt_1053
54. Body_578_sldprt_1054
55. Body_579_sldprt_1055
56. Body_580_sldprt_1056
57. Body_581_sldprt_1057
58. Body_582_sldprt_1058
59. Body_583_sldprt_1059
60. Body_584_sldprt_1060
61. Body_585_sldprt_1061
62. Body_586_sldprt_1062
63. Body_587_sldprt_1063
64. Body_588_sldprt_1064
65. Body_589_sldprt_1065
66. Body_590_sldprt_1066
67. Body_591_sldprt_1067
68. Body_592_sldprt_1068
69. Body_593_sldprt_1069
70. Body_594_sldprt_1070
71. Body_595_sldprt_1071
72. Body_596_sldprt_1072
73. Body_597_sldprt_1073
74. Body_598_sldprt_1074
75. Body_599_sldprt_1075
76. Body_600_sldprt_1076
77. Body_601_sldprt_1077
78. Body_602_sldprt_1078
79. Body_603_sldprt_1079
80. Body_604_sldprt_1080
81. Body_605_sldprt_1081
82. Body_606_sldprt_1082
83. Body_607_sldprt_1083
84. Body_608_sldprt_1084
85. Body_609_sldprt_1085
86. Body_610_sldprt_1086
87. Body_611_sldprt_1087
88. Body_612_sldprt_1088
89. Body_613_sldprt_1089
90. Body_614_sldprt_1090
91. Body_615_sldprt_1091
92. Body_616_sldprt_1092
93. Body_617_sldprt_1093
94. Body_618_sldprt_1094
95. Body_619_sldprt_1095
96. Body_620_sldprt_1096
97. Body_621_sldprt_1097
98. Body_622_sldprt_1098
99. Body_623_sldprt_1099
100. Body_624_sldprt_1100
101. Body_625_sldprt_1101
102. Body_626_sldprt_1102
103. Body_627_sldprt_1103
104. Body_628_sldprt_1104
105. Body_629_sldprt_1105
106. Body_630_sldprt_1106
107. Body_631_sldprt_1107
108. Body_632_sldprt_1108
109. Body_633_sldprt_1109
110. Body_634_sldprt_1110
111. Body_635_sldprt_1111
112. Body_636_sldprt_1112
113. Body_637_sldprt_1113
114. Body_638_sldprt_1114
115. Body_639_sldprt_1115
116. Body_640_sldprt_1116
117. Body_641_sldprt_1117
118. Body_642_sldprt_1118
119. Body_643_sldprt_1119
120. Body_644_sldprt_1120
121. Body_645_sldprt_1121
122. Body_646_sldprt_1122
123. Body_647_sldprt_1123
124. Body_648_sldprt_1124
125. Body_649_sldprt_1125
126. Body_650_sldprt_1126
127. Body_651_sldprt_1127
128. Body_652_sldprt_1128
129. Body_653_sldprt_1129
130. Body_654_sldprt_1130
131. Body_655_sldprt_1131
132. Body_656_sldprt_1132
133. Body_657_sldprt_1133
134. Body_658_sldprt_1134
135. Body_659_sldprt_1135
136. Body_660_sldprt_1136
137. Body_661_sldprt_1137
138. Body_662_sldprt_1138
139. Body_663_sldprt_1139
140. Body_664_sldprt_1140
141. Body_665_sldprt_1141
142. Body_666_sldprt_1142
143. Body_667_sldprt_1143
144. Body_668_sldprt_1144
145. Body_669_sldprt_1145
146. Body_670_sldprt_1146
147. Body_671_sldprt_1147
148. Body_672_sldprt_1148
149. Body_673_sldprt_1149
150. Body_674_sldprt_1150
151. Body_675_sldprt_1151
152. Body_676_sldprt_1152
153. Body_677_sldprt_1153
154. Body_678_sldprt_1154
155. Body_679_sldprt_1155
156. Body_680_sldprt_1156
157. Body_681_sldprt_1157
158. Body_682_sldprt_1158
159. Body_683_sldprt_1159
160. Body_684_sldprt_1160
161. Body_685_sldprt_1161
162. Body_686_sldprt_1162
163. Body_687_sldprt_1163
164. Body_688_sldprt_1164
165. Body_689_sldprt_1165
166. Body_690_sldprt_1166
167. Body_691_sldprt_1167
168. Body_692_sldprt_1168
169. Body_693_sldprt_1169
170. Body_694_sldprt_1170
171. Body_695_sldprt_1171
172. Body_696_sldprt_1172
173. Body_697_sldprt_1173
174. Body_698_sldprt_1174
175. Body_699_sldprt_1175
176. Body_700_sldprt_1176
177. Body_701_sldprt_1177
178. Body_702_sldprt_1178
179. Body_703_sldprt_1179
180. Body_704_sldprt_1180
181. Body_705_sldprt_1181
182. Body_706_sldprt_1182
183. Body_707_sldprt_1183
184. Body_708_sldprt_1184
185. Body_709_sldprt_1185
186. Body_710_sldprt_1186
187. Body_711_sldprt_1187
188. Body_712_sldprt_1188
189. Body_713_sldprt_1189
190. Body_714_sldprt_1190
191. Body_715_sldprt_1191
192. Body_716_sldprt_1192
193. Body_717_sldprt_1193
194. Body_718_sldprt_1194
195. Body_719_sldprt_1195
196. Body_720_sldprt_1196
197. Body_721_sldprt_1197
198. Body_722_sldprt_1198
199. Body_723_sldprt_1199
200. Body_724_sldprt_1200
201. Body_725_sldprt_1201
202. Body_726_sldprt_1202
203. Body_727_sldprt_1203
204. Body_728_sldprt_1204
205. Body_729_sldprt_1205
206. Body_730_sldprt_1206
207. Body_731_sldprt_1207
208. Body_732_sldprt_1208
209. Body_733_sldprt_1209
210. Body_734_sldprt_1210
211. Body_735_sldprt_1211
212. Body_736_sldprt_1212
213. Body_737_sldprt_1213
214. Body_738_sldprt_1214
215. Body_739_sldprt_1215
216. Body_740_sldprt_1216
217. Body_741_sldprt_1217
218. Body_742_sldprt_1218
219. Body_743_sldprt_1219
220. Body_744_sldprt_1220
221. Body_745_sldprt_1221
222. Body_746_sldprt_1222
223. Body_747_sldprt_1223
224. Body_748_sldprt_1224
225. Body_749_sldprt_1225
226. Body_750_sldprt_1226
227. Body_751_sldprt_1227
228. Body_752_sldprt_1228
229. Body_753_sldprt_1229
230. Body_754_sldprt_1230
231. Body_755_sldprt_1231
232. Body_756_sldprt_1232
233. Body_757_sldprt_1233
234. Body_758_sldprt_1234
235. Body_759_sldprt_1235
236. Body_760_sldprt_1236
237. Body_761_sldprt_1237
238. Body_762_sldprt_1238
239. Body_763_sldprt_1239
240. Body_764_sldprt_1240
241. Body_765_sldprt_1241
242. Body_766_sldprt_1242
243. Body_767_sldprt_1243
244. Body_768_sldprt_1244
245. Body_769_sldprt_1245
246. Body_770_sldprt_1246
247. Body_771_sldprt_1247
248. Body_772_sldprt_1248
249. Body_773_sldprt_1249
250. Body_774_sldprt_1250
251. Body_775_sldprt_1251
252. Body_776_sldprt_1252
253. Body_777_sldprt_1253
254. Body_778_sldprt_1254
255. Body_779_sldprt_1255
256. Body_780_sldprt_1256
257. Body_781_sldprt_1257
258. Body_782_sldprt_1258
259. Body_783_sldprt_1259
260. Body_784_sldprt_1260
261. Body_785_sldprt_1261
262. Body_786_sldprt_1262
263. Body_787_sldprt_1263
264. Body_788_sldprt_1264
265. Body_789_sldprt_1265
266. Body_790_sldprt_1266
267. Body_791_sldprt_1267
268. Body_792_sldprt_1268